# Autodesk Inventor assembly: driven wheel assembly right
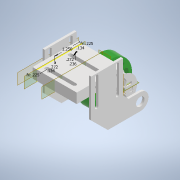
[picture p0: Inventor's stored thumbnail of the model, 180x180]
Saved by Autodesk Inventor 2020 (Build 240168000, 168)
## iProperties
Created: 2020-01-25
Part Number: driven wheel assembly right
Document SubType Name: Assembly
Designer: ball
Author: ball
## Documents named in this file (4)
- D:\FTC8863\2019 Robot\Collection\Intake\driven wheel assembly right.iam
- D:\FTC8863\2019 Robot\Collection\Intake\driven wheel mount to xrail.ipt
- D:\FTC8863\2019 Robot\general robot componets\pulley .25 in + wheel.2.iam
- D:\FTC8863\2019 Robot\Collection\Intake\driven wheel arm angled.ipt
## Components (4 placed, 3 different names)
1. driven wheel mount to xrail:1 — Flush:1, Flush:2, Mate:1
2. driven wheel arm angled:1 — Flush:1, Flush:2, Flush:3, Mate:2, Mate:3
3. pulley .25 in + wheel.2:1 [sub-assembly] — Mate:3, Mate:4
4. driven wheel arm angled:2 — Mate:1, Flush:3, Mate:2, Mate:4
## Relationships (7: Mate 4, Flush 3)
- Flush:1: driven wheel mount to xrail:1 ↔ driven wheel arm angled:1
- Flush:2: driven wheel mount to xrail:1 ↔ driven wheel arm angled:1
- Mate:1: driven wheel mount to xrail:1 ↔ driven wheel arm angled:2
- Flush:3: driven wheel arm angled:1 ↔ driven wheel arm angled:2
- Mate:2: driven wheel arm angled:1 ↔ driven wheel arm angled:2
- Mate:3: driven wheel arm angled:1 ↔ pulley .25 in + wheel.2:1
- Mate:4 (6.35 mm): pulley .25 in + wheel.2:1 ↔ driven wheel arm angled:2
